# Autodesk Inventor assembly: 人孔
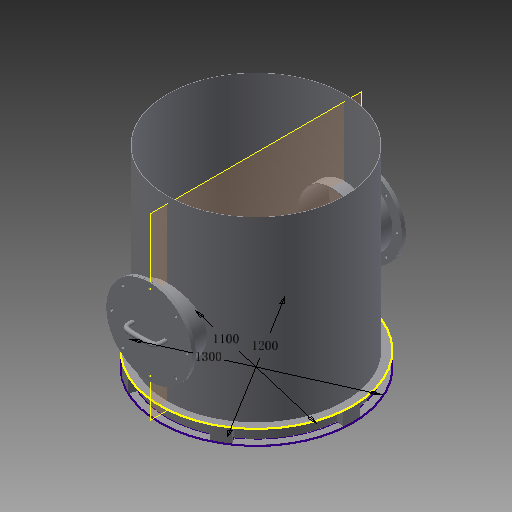
[picture p0: Inventor's stored thumbnail of the model, 512x512]
Saved by Autodesk Inventor 2018.2 (Build 222227000, 227)
## iProperties
Created: 2018-07-04
Part Number: 人孔
Material: 常规
Document SubType Name: Assembly
Designer: Administrator
Author: Administrator
## Documents named in this file (5)
- C:\Users\Administrator\Desktop\填料塔\结构件1.iam
- C:\Users\Administrator\Desktop\填料塔\人孔法兰.ipt
- C:\Users\Administrator\Desktop\填料塔\人孔.ipt
- C:\Users\Administrator\Desktop\人孔\设计加速器\螺栓联接2.iam
- C:\Users\Administrator\Desktop\填料塔\裙座.ipt
## Components (6 placed, 4 different names)
1. 人孔法兰:1 — 旋转:1
2. 人孔:1 — 旋转:1, 圆柱:1
3. 螺栓联接:1 [sub-assembly]
4. 裙座:1 — 表面齐平:1, 圆柱:1, 圆柱:2
5. 人孔法兰:2
6. 人孔:2 — 圆柱:2
## Relationships (5: RevoluteJoint 2, CylindricalJoint 2, Flush 1)
- 旋转:1 [RevoluteJoint]: 人孔法兰:1 ↔ 人孔:1
- [RevoluteJoint]: 人孔法兰:2 ↔ 人孔:2
- 表面齐平:1 [Flush]: 裙座:1
- 圆柱:1 [CylindricalJoint]: 人孔:1 ↔ 裙座:1
- 圆柱:2 [CylindricalJoint]: 裙座:1 ↔ 人孔:2
## Named parameters: d7_d0 = 0 mm, d8_d1 = 90 deg
